# Autodesk Inventor assembly: HoodGear
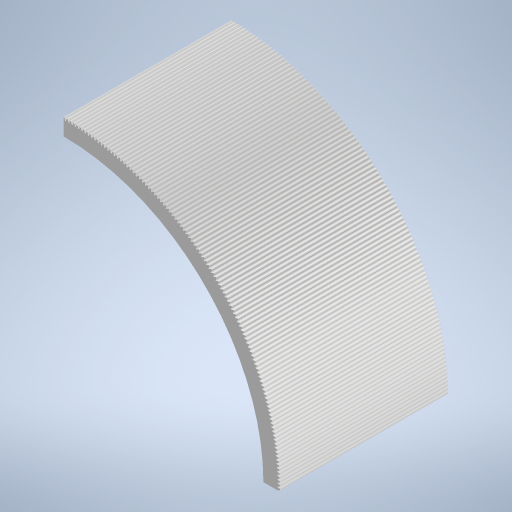
[picture p0: Inventor's stored thumbnail of the model, 512x512]
Saved by Autodesk Inventor 2023.3 (Build 273359000, 359)
## iProperties
Created: 2023-11-15
Part Number: HoodGear
Document SubType Name: Assembly
Designer: jackc
Author: jackc
## Documents named in this file (4)
- C:\Users\jackc\OneDrive\CAD\Parametric Turret\Gears and Pulleys\HoodGear.iam
- C:\Users\jackc\OneDrive\CAD\Parametric Turret\Gears and Pulleys\HoodGearSmooth.ipt
- C:\Users\jackc\OneDrive\CAD\Parametric Turret\Parameters.ipt
- C:\Users\jackc\OneDrive\CAD\Parametric Turret\Gears and Pulleys\HoodGear\Design Accelerator\Spur Gears1.iam
## Components (2 placed, 2 different names)
1. HoodGearSmooth:1
2. Spur Gears:1 [sub-assembly]
## Named parameters: WheelSize = 101.6 mm, BallSize = 203.2 mm, Compression = 12.7 mm, TeethNumber = 410
